# Autodesk Inventor assembly: s-assy-linear_joint
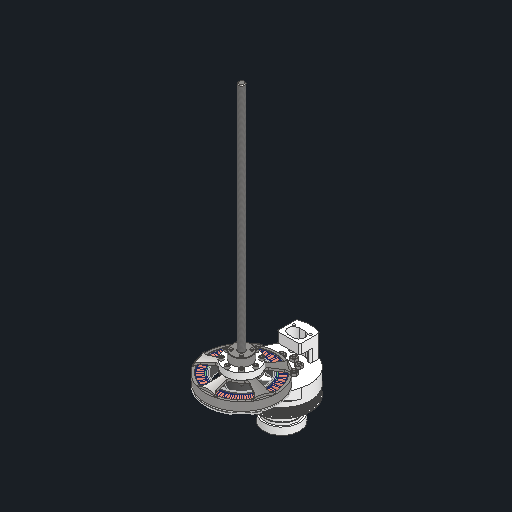
[picture p0: Inventor's stored thumbnail of the model, 512x512]
Saved by Autodesk Inventor 2022 (Build 260153000, 153)
## iProperties
Created: 2021-10-11
Part Number: s-assy-linear_joint
Document SubType Name: Assembly
Designer: Yuta Kage
Mass: 635.308 g
Surface Area: 1163.48 cm^2
Volume: 204.408 cm^3
Density: 3.10804 g/cm^3
Author: Yuta Kage
## Documents named in this file (18)
- C:\Users\yuta0\Documents\GitHub\catchrobo_hardware\assy-scara\s-assy-linear_joint.iam
- C:\Users\yuta0\Documents\GitHub\catchrobo_hardware\assy-scara\lead_screw.ipt
- C:\Users\yuta0\Documents\GitHub\catchrobo_hardware\assy-scara\ex8108.iam
- C:\Users\yuta0\Documents\GitHub\catchrobo_hardware\assy-scara\SCSTR8-10.iam
- C:\Users\yuta0\Documents\GitHub\catchrobo_hardware\assy-scara\scara-base10.ipt
- C:\Users\yuta0\Documents\GitHub\catchrobo_hardware\assy-scara\CB3-15.ipt
- C:\Users\yuta0\Documents\GitHub\catchrobo_hardware\assy-scara\C-LMUW8.ipt
- C:\Users\yuta0\Documents\GitHub\catchrobo_hardware\assy-scara\scara-base16.ipt
- C:\Users\yuta0\Documents\GitHub\catchrobo_hardware\assy-scara\scara-base20.ipt
- C:\Users\yuta0\Documents\GitHub\catchrobo_hardware\assy-scara\CB2-4.ipt
- C:\Users\yuta0\Documents\GitHub\catchrobo_hardware\assy-scara\SB-203040.ipt
- C:\Users\yuta0\Documents\GitHub\catchrobo_hardware\assy-scara\s-assy-AS5047P-TS_EK_AB.iam
- C:\Users\yuta0\Documents\GitHub\catchrobo_hardware\assy-scara\CB4-10.ipt
- C:\Users\yuta0\Documents\GitHub\catchrobo_hardware\assy-scara\s-assy-scara-magnet.iam
- C:\Users\yuta0\Documents\GitHub\catchrobo_hardware\assy-scara\CB4-60.ipt
- C:\Users\yuta0\Documents\GitHub\catchrobo_hardware\assy-scara\LBNR4.ipt
- C:\Users\yuta0\Documents\GitHub\catchrobo_hardware\assy-scara\CB4-15.ipt
- C:\Users\yuta0\Documents\GitHub\catchrobo_hardware\assy-scara\scara-base13.ipt
## Components (51 placed, 17 different names)
1. lead_screw:1 — メイト:1, メイト:5, フラッシュ:1
2. ex8108:1 [sub-assembly] — メイト:1, メイト:2, メイト:3, メイト:4, メイト:50, メイト:51, メイト:52, メイト:53, メイト:88, メイト:89, メイト:90
3. SCSTR8-10:1 [sub-assembly] — メイト:5, メイト:6, メイト:7
4. scara-base10:1 — メイト:2, メイト:3, メイト:4, メイト:6, メイト:7, メイト:12, メイト:13, フラッシュ:1, メイト:16, メイト:17
5. C-LMUW8:3 — メイト:85, メイト:86
6. s-assy-scara-magnet:1 [sub-assembly] — メイト:50, メイト:51, メイト:52, メイト:53
7. scara-base16:1 — メイト:66, メイト:83, メイト:86, メイト:87, メイト:106
8. scara-base20:2 — メイト:83, メイト:84, メイト:85, メイト:87, メイト:88, メイト:89, メイト:90, メイト:91, メイト:92, メイト:95, メイト:100, メイト:101, メイト:103, メイト:104, メイト:105, メイト:107, メイト:108, メイト:109
9. s-assy-AS5047P-TS_EK_AB:1 [sub-assembly] — メイト:95, メイト:96, メイト:97, メイト:98, メイト:99
10. scara-base13:1 — メイト:107, メイト:108, メイト:109
11. CB4-15:1 — メイト:12, メイト:13
12. CB4-15:2
13. CB4-15:3
14. CB3-15:4 — メイト:16, メイト:17
15. CB3-15:5
16. CB3-15:6
17. CB3-15:7
18. CB3-15:8
19. CB3-15:9
20. CB3-15:10
21. CB3-15:11
22. CB4-60:1 — メイト:66, メイト:102, メイト:106
23. LBNR4:1 — メイト:102, メイト:103
24. CB4-60:2
25. LBNR4:2
26. CB4-60:3
27. LBNR4:3
28. CB4-60:4 — メイト:84
29. LBNR4:4
30. CB4-60:5
31. LBNR4:5
32. CB4-60:6
33. LBNR4:6
34. CB4-60:7
35. LBNR4:7
36. CB4-60:8
37. LBNR4:8
38. SB-203040:1 — メイト:91, メイト:92, メイト:97
39. CB2-4:1 — メイト:98, メイト:99
40. SB-203040:2
41. CB2-4:2
42. SB-203040:3 — メイト:96
43. CB2-4:3
44. SB-203040:4
45. CB2-4:4
46. CB4-10:1 — メイト:100, メイト:101
47. CB4-10:2
48. CB4-10:3
49. CB4-10:4
50. CB3-15:12 — メイト:104, メイト:105
51. CB3-15:13
## Component patterns: (3 elements, first: CB4-15:1), (8 elements, first: CB3-15:4), (8 elements, first: CB4-60:1 + LBNR4:1), (4 elements, first: SB-203040:1 + CB2-4:1), (4 elements, first: CB4-10:1), (2 elements, first: CB3-15:12)
## Relationships (42: Mate 41, Flush 1)
- メイト:1 [Mate]: lead_screw:1 ↔ ex8108:1
- メイト:2 [Mate]: ex8108:1 ↔ scara-base10:1
- メイト:3 [Mate]: ex8108:1 ↔ scara-base10:1
- メイト:4 [Mate]: ex8108:1 ↔ scara-base10:1
- メイト:5 [Mate]: lead_screw:1 ↔ SCSTR8-10:1
- メイト:6 [Mate]: SCSTR8-10:1 ↔ scara-base10:1
- メイト:7 [Mate]: SCSTR8-10:1 ↔ scara-base10:1
- メイト:12 [Mate]: scara-base10:1 ↔ CB4-15:1
- メイト:13 [Mate]: scara-base10:1 ↔ CB4-15:1
- フラッシュ:1 [Flush]: lead_screw:1 ↔ scara-base10:1
- メイト:16 [Mate]: scara-base10:1 ↔ CB3-15:4
- メイト:17 [Mate]: scara-base10:1 ↔ CB3-15:4
- メイト:50 [Mate]: ex8108:1 ↔ s-assy-scara-magnet:1
- メイト:51 [Mate]: ex8108:1 ↔ s-assy-scara-magnet:1
- メイト:52 [Mate]: ex8108:1 ↔ s-assy-scara-magnet:1
- メイト:53 [Mate]: ex8108:1 ↔ s-assy-scara-magnet:1
- メイト:66 [Mate]: scara-base16:1 ↔ CB4-60:1
- メイト:83 [Mate]: scara-base16:1 ↔ scara-base20:2
- メイト:84 [Mate]: scara-base20:2 ↔ CB4-60:4
- メイト:85 [Mate]: C-LMUW8:3 ↔ scara-base20:2
- メイト:86 [Mate]: C-LMUW8:3 ↔ scara-base16:1
- メイト:87 [Mate]: scara-base16:1 ↔ scara-base20:2
- メイト:88 [Mate]: ex8108:1 ↔ scara-base20:2
- メイト:89 [Mate]: ex8108:1 ↔ scara-base20:2
- メイト:90 [Mate]: ex8108:1 ↔ scara-base20:2
- メイト:91 [Mate]: scara-base20:2 ↔ SB-203040:1
- メイト:92 [Mate]: scara-base20:2 ↔ SB-203040:1
- メイト:95 [Mate]: scara-base20:2 ↔ s-assy-AS5047P-TS_EK_AB:1
- メイト:96 [Mate]: s-assy-AS5047P-TS_EK_AB:1 ↔ SB-203040:3
- メイト:97 [Mate]: s-assy-AS5047P-TS_EK_AB:1 ↔ SB-203040:1
- メイト:98 [Mate]: s-assy-AS5047P-TS_EK_AB:1 ↔ CB2-4:1
- メイト:99 [Mate]: s-assy-AS5047P-TS_EK_AB:1 ↔ CB2-4:1
- メイト:100 [Mate]: scara-base20:2 ↔ CB4-10:1
- メイト:101 [Mate]: scara-base20:2 ↔ CB4-10:1
- メイト:102 [Mate]: CB4-60:1 ↔ LBNR4:1
- メイト:103 [Mate]: scara-base20:2 ↔ LBNR4:1
- メイト:104 [Mate]: scara-base20:2 ↔ CB3-15:12
- メイト:105 [Mate]: scara-base20:2 ↔ CB3-15:12
- メイト:106 [Mate]: scara-base16:1 ↔ CB4-60:1
- メイト:107 [Mate]: scara-base20:2 ↔ scara-base13:1
- メイト:108 [Mate]: scara-base20:2 ↔ scara-base13:1
- メイト:109 [Mate]: scara-base20:2 ↔ scara-base13:1
